# Autodesk Inventor assembly: ASSEMBLY_Main
(part 3 of 4)
- Równoległy:93 [Flush] (2 mm): COTS_GENERIC_20x40mm_alu_extrusion_560mm:1 ↔ LCBN_ALU_2mm_Y_Axis_Motor_Mount:1
- Zestawiający:100 [Mate]: COTS_GENERIC_Bearing_12x5x5:1 ↔ COTS_GENERIC_Y_Axis_Timing_Belt:1
- Zestawiający:101 [Mate]: COTS_GENERIC_NEMA23_Stepper_Motor:1 ↔ COTS_GENERIC_Y_Axis_Timing_Belt:1
- Zestawiający:102 [Mate] (0.5 mm): COTS_GENERIC_NEMA23_Stepper_Motor:1 ↔ COTS_GENERIC_Y_Axis_Timing_Belt:1
- Zestawiający:103 [Mate] (1 mm): COTS_GENERIC_Bearing_12x5x5:1 ↔ COTS_GENERIC_22x5_Washer:2
- Zestawiający:104 [Mate] (1 mm): COTS_GENERIC_Bearing_12x5x5:2 ↔ COTS_GENERIC_22x5_Washer:1
- Zestawiający:107 [Mate]: LCBN_ALU_3mm_Y_Axis_Idler_Stiffener_Top:1 ↔ COTS_GENERIC_22x5_Washer:2
- Zestawiający:108 [Mate]: LCBN_STEEL_3mm_Y_Axis_Heatbed_Baseplate:1 ↔ 3DP_ABS_Y_Axis_Linear_Bearing_Mount_Top:1
- Zestawiający:109 [Mate]: LCBN_STEEL_3mm_Y_Axis_Heatbed_Baseplate:1 ↔ 3DP_ABS_Y_Axis_Linear_Bearing_Mount_Top:4
- Zestawiający:110 [Mate]: LCBN_STEEL_3mm_Y_Axis_Heatbed_Baseplate:1 ↔ 3DP_ABS_Y_Axis_Linear_Bearing_Mount_Top:3
- Zestawiający:111 [Mate]: LCBN_STEEL_3mm_Y_Axis_Heatbed_Baseplate:1 ↔ 3DP_ABS_Y_Axis_Linear_Bearing_Mount_Top:2
- Zestawiający:112 [Mate]: LCBN_STEEL_3mm_Y_Axis_Heatbed_Baseplate:1 ↔ 3DP_ABS_Y_Axis_Linear_Bearing_Mount_Top:1
- Zestawiający:113 [Mate]: LCBN_STEEL_3mm_Y_Axis_Heatbed_Baseplate:1 ↔ 3DP_ABS_Y_Axis_Linear_Bearing_Mount_Top:1
- Zestawiający:114 [Mate]: LCBN_STEEL_3mm_Y_Axis_Heatbed_Baseplate:1 ↔ 3DP_ABS_Y_Axis_Linear_Bearing_Mount_Top:4
- Zestawiający:115 [Mate]: LCBN_STEEL_3mm_Y_Axis_Heatbed_Baseplate:1 ↔ 3DP_ABS_Y_Axis_Linear_Bearing_Mount_Top:4
- Zestawiający:116 [Mate]: LCBN_STEEL_3mm_Y_Axis_Heatbed_Baseplate:1 ↔ 3DP_ABS_Y_Axis_Linear_Bearing_Mount_Top:3
- Zestawiający:117 [Mate]: LCBN_STEEL_3mm_Y_Axis_Heatbed_Baseplate:1 ↔ 3DP_ABS_Y_Axis_Linear_Bearing_Mount_Top:3
- Zestawiający:118 [Mate]: LCBN_STEEL_3mm_Y_Axis_Heatbed_Baseplate:1 ↔ 3DP_ABS_Y_Axis_Linear_Bearing_Mount_Top:2
- Zestawiający:119 [Mate]: LCBN_STEEL_3mm_Y_Axis_Heatbed_Baseplate:1 ↔ 3DP_ABS_Y_Axis_Linear_Bearing_Mount_Top:2
- Zestawiający:120 [Mate] (1 mm): 3DP_ABS_Y_Axis_Linear_Bearing_Mount_Top:3 ↔ 3DP_ABS_Y_Axis_Linear_Bearing_Mount_Bottom:1
- Zestawiający:121 [Mate] (1 mm): 3DP_ABS_Y_Axis_Linear_Bearing_Mount_Top:2 ↔ 3DP_ABS_Y_Axis_Linear_Bearing_Mount_Bottom:3
- Zestawiający:122 [Mate] (1 mm): 3DP_ABS_Y_Axis_Linear_Bearing_Mount_Top:4 ↔ 3DP_ABS_Y_Axis_Linear_Bearing_Mount_Bottom:2
- Zestawiający:123 [Mate] (1 mm): 3DP_ABS_Y_Axis_Linear_Bearing_Mount_Top:1 ↔ 3DP_ABS_Y_Axis_Linear_Bearing_Mount_Bottom:4
- Równoległy:94 [Flush]: 3DP_ABS_Y_Axis_Linear_Bearing_Mount_Top:1 ↔ 3DP_ABS_Y_Axis_Linear_Bearing_Mount_Bottom:4
- Równoległy:95 [Flush] (3 mm): 3DP_ABS_Y_Axis_Linear_Bearing_Mount_Top:1 ↔ 3DP_ABS_Y_Axis_Linear_Bearing_Mount_Bottom:4
- Równoległy:96 [Flush]: 3DP_ABS_Y_Axis_Linear_Bearing_Mount_Top:4 ↔ 3DP_ABS_Y_Axis_Linear_Bearing_Mount_Bottom:2
- Równoległy:97 [Flush] (3 mm): 3DP_ABS_Y_Axis_Linear_Bearing_Mount_Top:4 ↔ 3DP_ABS_Y_Axis_Linear_Bearing_Mount_Bottom:2
- Równoległy:98 [Flush]: 3DP_ABS_Y_Axis_Linear_Bearing_Mount_Top:2 ↔ 3DP_ABS_Y_Axis_Linear_Bearing_Mount_Bottom:3
- Równoległy:99 [Flush] (3 mm): 3DP_ABS_Y_Axis_Linear_Bearing_Mount_Top:2 ↔ 3DP_ABS_Y_Axis_Linear_Bearing_Mount_Bottom:3
- Równoległy:100 [Flush]: 3DP_ABS_Y_Axis_Linear_Bearing_Mount_Top:3 ↔ 3DP_ABS_Y_Axis_Linear_Bearing_Mount_Bottom:1
- Równoległy:101 [Flush] (3 mm): 3DP_ABS_Y_Axis_Linear_Bearing_Mount_Top:3 ↔ 3DP_ABS_Y_Axis_Linear_Bearing_Mount_Bottom:1
- Zestawiający:124 [Mate]: COTS_GENERIC_LM10UU_10mm_Linear_Bearing:3 ↔ 3DP_ABS_Y_Axis_Linear_Bearing_Mount_Top:2
- Zestawiający:125 [Mate]: CUT_STEEL_10mmx457mm_Linear_Shaft:2 ↔ 3DP_ABS_Y_Axis_Linear_Bearing_Mount_Top:4
- Zestawiający:126 [Mate] (0.25 mm): COTS_GENERIC_LM10UU_10mm_Linear_Bearing:2 ↔ 3DP_ABS_Y_Axis_Linear_Bearing_Mount_Top:4
- Zestawiający:127 [Mate] (0.25 mm): COTS_GENERIC_LM10UU_10mm_Linear_Bearing:3 ↔ 3DP_ABS_Y_Axis_Linear_Bearing_Mount_Top:2
- Zestawiający:128 [Mate] (0.25 mm): COTS_GENERIC_LM10UU_10mm_Linear_Bearing:1 ↔ 3DP_ABS_Y_Axis_Linear_Bearing_Mount_Top:1
- Zestawiający:129 [Mate] (0.25 mm): COTS_GENERIC_LM10UU_10mm_Linear_Bearing:4 ↔ 3DP_ABS_Y_Axis_Linear_Bearing_Mount_Top:3
- Zestawiający:130 [Mate]: LCBN_STEEL_3mm_Y_Axis_Heatbed_Baseplate:1 ↔ 3DP_ABS_Y_Axis_Belt_Mount_Spacer:1
- Zestawiający:131 [Mate]: LCBN_STEEL_3mm_Y_Axis_Heatbed_Baseplate:1 ↔ 3DP_ABS_Y_Axis_Belt_Mount_Spacer:2
- Zestawiający:132 [Mate]: LCBN_STEEL_3mm_Y_Axis_Heatbed_Baseplate:1 ↔ 3DP_ABS_Y_Axis_Belt_Mount_Spacer:1
- Zestawiający:133 [Mate]: LCBN_STEEL_3mm_Y_Axis_Heatbed_Baseplate:1 ↔ 3DP_ABS_Y_Axis_Belt_Mount_Spacer:2
- Równoległy:102 [Flush] (2.5 mm): LCBN_STEEL_3mm_Y_Axis_Heatbed_Baseplate:1 ↔ 3DP_ABS_Y_Axis_Belt_Mount_Spacer:1
- Równoległy:103 [Flush] (2.5 mm): LCBN_STEEL_3mm_Y_Axis_Heatbed_Baseplate:1 ↔ 3DP_ABS_Y_Axis_Belt_Mount_Spacer:2
- Zestawiający:134 [Mate]: COTS_GENERIC_SMA12GUU_Linear_Bearing_Block:2 ↔ LC_ALU_4mm_X_End_Motor_Side:1
- Zestawiający:135 [Mate] (3 mm): COTS_GENERIC_NEMA17_25mm_shaft:1 ↔ LC_ALU_4mm_X_End_Motor_Side:1
- Równoległy:104 [Flush]: COTS_GENERIC_SMA12GUU_Linear_Bearing_Block:2 ↔ LC_ALU_4mm_X_End_Motor_Side:1
- Równoległy:105 [Flush]: COTS_GENERIC_SMA12GUU_Linear_Bearing_Block:4 ↔ LC_ALU_4mm_X_End_Motor_Side:1
- Równoległy:106 [Flush]: COTS_GENERIC_SMA12GUU_Linear_Bearing_Block:2 ↔ LC_ALU_4mm_X_End_Motor_Side:1
- Zestawiający:137 [Mate]: LC_ALU_4mm_X_End_Motor_Side:1 ↔ 3DP_ABS_X_Axis_Linear_Shaft_Clamp_Base:1
- Zestawiający:138 [Mate]: LC_ALU_4mm_X_End_Motor_Side:1 ↔ 3DP_ABS_X_Axis_Linear_Shaft_Clamp_Base:2
- Równoległy:107 [Flush]: LC_ALU_4mm_X_End_Motor_Side:1 ↔ 3DP_ABS_X_Axis_Linear_Shaft_Clamp_Base:1
- Równoległy:108 [Flush]: LC_ALU_4mm_X_End_Motor_Side:1 ↔ 3DP_ABS_X_Axis_Linear_Shaft_Clamp_Base:1
- Równoległy:109 [Flush]: LC_ALU_4mm_X_End_Motor_Side:1 ↔ 3DP_ABS_X_Axis_Linear_Shaft_Clamp_Base:2
- Równoległy:110 [Flush]: LC_ALU_4mm_X_End_Motor_Side:1 ↔ 3DP_ABS_X_Axis_Linear_Shaft_Clamp_Base:2
- Zestawiający:139 [Mate]: CUT_STEEL_10mmx516mm_Linear_Shaft:1 ↔ 3DP_ABS_X_Axis_Linear_Shaft_Clamp_Base:2
- Zestawiający:140 [Mate]: CUT_STEEL_10mmx516mm_Linear_Shaft:2 ↔ 3DP_ABS_X_Axis_Linear_Shaft_Clamp_Base:1
- Równoległy:111 [Flush]: CUT_STEEL_10mmx516mm_Linear_Shaft:1 ↔ 3DP_ABS_X_Axis_Linear_Shaft_Clamp_Base:2
- Równoległy:112 [Flush]: CUT_STEEL_10mmx516mm_Linear_Shaft:2 ↔ 3DP_ABS_X_Axis_Linear_Shaft_Clamp_Base:1
- Zestawiający:141 [Mate]: ASSEMBLY_X_Axis_Carriage_and_Extruder_Belt_Gearbox:1 ↔ CUT_STEEL_10mmx516mm_Linear_Shaft:2
- Zestawiający:142 [Mate] (-12 mm): ASSEMBLY_X_Axis_Carriage_and_Extruder_Belt_Gearbox:1 ↔ CUT_STEEL_10mmx516mm_Linear_Shaft:1
- Zestawiający:143 [Mate]: COTS_GENERIC_SMA12GUU_Linear_Bearing_Block:3 ↔ LC_ALU_4mm_X_End_Bearing_Side:1
- Równoległy:113 [Flush]: COTS_GENERIC_SMA12GUU_Linear_Bearing_Block:1 ↔ LC_ALU_4mm_X_End_Bearing_Side:1
- Równoległy:114 [Flush]: COTS_GENERIC_SMA12GUU_Linear_Bearing_Block:1 ↔ LC_ALU_4mm_X_End_Bearing_Side:1
- Zestawiający:144 [Mate]: LC_ALU_4mm_X_End_Bearing_Side:1 ↔ 3DP_ABS_X_Axis_Linear_Shaft_Clamp_Base:3
- Zestawiający:145 [Mate]: LC_ALU_4mm_X_End_Bearing_Side:1 ↔ 3DP_ABS_X_Axis_Linear_Shaft_Clamp_Base:4
- Równoległy:115 [Flush]: LC_ALU_4mm_X_End_Bearing_Side:1 ↔ 3DP_ABS_X_Axis_Linear_Shaft_Clamp_Base:4
- Równoległy:116 [Flush]: LC_ALU_4mm_X_End_Bearing_Side:1 ↔ 3DP_ABS_X_Axis_Linear_Shaft_Clamp_Base:3
- Równoległy:117 [Flush]: LC_ALU_4mm_X_End_Bearing_Side:1 ↔ 3DP_ABS_X_Axis_Linear_Shaft_Clamp_Base:4
- Równoległy:118 [Flush]: LC_ALU_4mm_X_End_Bearing_Side:1 ↔ 3DP_ABS_X_Axis_Linear_Shaft_Clamp_Base:3
- Zestawiający:146 [Mate] (1 mm): 3DP_ABS_X_Axis_Linear_Shaft_Clamp_Base:1 ↔ 3DP_ABS_X_Axis_Linear_Shaft_Clamp_Top:2
- Równoległy:119 [Flush]: 3DP_ABS_X_Axis_Linear_Shaft_Clamp_Base:1 ↔ 3DP_ABS_X_Axis_Linear_Shaft_Clamp_Top:2
- Równoległy:120 [Flush]: 3DP_ABS_X_Axis_Linear_Shaft_Clamp_Base:1 ↔ 3DP_ABS_X_Axis_Linear_Shaft_Clamp_Top:2
- Zestawiający:147 [Mate] (1 mm): 3DP_ABS_X_Axis_Linear_Shaft_Clamp_Base:3 ↔ 3DP_ABS_X_Axis_Linear_Shaft_Clamp_Top:1
- Równoległy:121 [Flush]: 3DP_ABS_X_Axis_Linear_Shaft_Clamp_Base:3 ↔ 3DP_ABS_X_Axis_Linear_Shaft_Clamp_Top:1
- Równoległy:122 [Flush]: 3DP_ABS_X_Axis_Linear_Shaft_Clamp_Base:3 ↔ 3DP_ABS_X_Axis_Linear_Shaft_Clamp_Top:1
- Zestawiający:149 [Mate]: 3DP_ABS_X_Axis_Linear_Shaft_Clamp_Base:4 ↔ 3DP_ABS_X_Axis_Linear_Shaft_Clamp_Bottom:2
- Równoległy:123 [Flush]: 3DP_ABS_X_Axis_Linear_Shaft_Clamp_Base:4 ↔ 3DP_ABS_X_Axis_Linear_Shaft_Clamp_Bottom:2
- Równoległy:124 [Flush]: 3DP_ABS_X_Axis_Linear_Shaft_Clamp_Base:4 ↔ 3DP_ABS_X_Axis_Linear_Shaft_Clamp_Bottom:2
- Zestawiający:152 [Mate]: COTS_GENERIC_20x40mm_alu_extrusion_460mm:1 ↔ 3DP_PLA_Controller_Case_Bottom:1
- Równoległy:128 [Flush]: COTS_GENERIC_20x40mm_alu_extrusion_560mm:1 ↔ 3DP_PLA_Controller_Case_Bottom:1
- Równoległy:129 [Flush]: COTS_GENERIC_20x40mm_alu_extrusion_460mm:1 ↔ 3DP_PLA_Controller_Case_Bottom:1
- Zestawiający:154 [Mate]: 3DP_PLA_Controller_Case_Bottom:1 ↔ 3DP_PLA_Controller_Case_Side_Wall_Longer:1
- Równoległy:130 [Flush]: 3DP_PLA_Controller_Case_Bottom:1 ↔ 3DP_PLA_Controller_Case_Side_Wall_Longer:1
- Równoległy:131 [Flush]: 3DP_PLA_Controller_Case_Bottom:1 ↔ 3DP_PLA_Controller_Case_Side_Wall_Longer:1
- Zestawiający:155 [Mate]: 3DP_PLA_Controller_Case_Bottom:1 ↔ 3DP_PLA_Controller_Case_Side_Wall_Shorter:1
- Równoległy:132 [Flush]: 3DP_PLA_Controller_Case_Bottom:1 ↔ 3DP_PLA_Controller_Case_Side_Wall_Shorter:1
- Równoległy:133 [Flush]: 3DP_PLA_Controller_Case_Bottom:1 ↔ 3DP_PLA_Controller_Case_Side_Wall_Shorter:1
- Zestawiający:156 [Mate]: COTS_GENERIC_RAMPS_14_Ardunio_Mega:1 ↔ 3DP_PLA_Controller_Case_Bottom:1
- Zestawiający:157 [Mate]: 3DP_PLA_Controller_Case_Side_Wall_Longer:1 ↔ 3DP_PLA_Controller_Case_Top:1
- Równoległy:134 [Flush]: COTS_GENERIC_20x40mm_alu_extrusion_460mm:1 ↔ 3DP_PLA_Controller_Case_Top:1
- Równoległy:135 [Flush]: COTS_GENERIC_20x40mm_alu_extrusion_560mm:1 ↔ 3DP_PLA_Controller_Case_Top:1
- Zestawiający:158 [Mate]: COTS_GENERIC_80mm_fan:1 ↔ 3DP_PLA_Controller_Case_Top:1
- Zestawiający:159 [Mate]: COTS_GENERIC_80mm_fan:1 ↔ 3DP_PLA_Controller_Case_Top:1
- Zestawiający:160 [Mate]: COTS_GENERIC_80mm_fan:1 ↔ 3DP_PLA_Controller_Case_Top:1
- Zestawiający:161 [Mate]: COTS_GENERIC_80mm_fan:1 ↔ 3DP_PLA_Controller_Case_Fan_Grill:1
- Zestawiający:162 [Mate]: COTS_GENERIC_80mm_fan:1 ↔ 3DP_PLA_Controller_Case_Fan_Grill:1
- Zestawiający:163 [Mate]: COTS_GENERIC_80mm_fan:1 ↔ 3DP_PLA_Controller_Case_Fan_Grill:1
- Zestawiający:164 [Mate]: COTS_GENERIC_20x40mm_alu_extrusion_560mm:2 ↔ 3DP_PLA_Filament_Spool_Rollers:2
- Zestawiający:165 [Mate]: COTS_GENERIC_20x40mm_alu_extrusion_560mm:2 ↔ 3DP_PLA_Filament_Spool_Rollers:1
- Równoległy:136 [Flush] (235 mm): COTS_GENERIC_20x40mm_alu_extrusion_460mm:3 ↔ 3DP_PLA_Filament_Spool_Rollers:1
- Zestawiający:166 [Mate] (1 mm): 3DP_PLA_Filament_Spool_Rollers:1 ↔ COTS_GENERIC_Bearing_19x5x6:1
- Zestawiający:167 [Mate] (1 mm): 3DP_PLA_Filament_Spool_Rollers:1 ↔ COTS_GENERIC_Bearing_19x5x6:2
- Zestawiający:168 [Mate] (1 mm): 3DP_PLA_Filament_Spool_Rollers:2 ↔ COTS_GENERIC_Bearing_19x5x6:4
- Zestawiający:169 [Mate] (1 mm): 3DP_PLA_Filament_Spool_Rollers:2 ↔ COTS_GENERIC_Bearing_19x5x6:3
- Zestawiający:170 [Mate]: 3DP_PLA_Filament_Spool_Rollers:1 ↔ COTS_GENERIC_Bearing_19x5x6:1
- Zestawiający:171 [Mate]: 3DP_PLA_Filament_Spool_Rollers:1 ↔ COTS_GENERIC_Bearing_19x5x6:2
- Zestawiający:172 [Mate]: 3DP_PLA_Filament_Spool_Rollers:2 ↔ COTS_GENERIC_Bearing_19x5x6:4
- Zestawiający:173 [Mate]: 3DP_PLA_Filament_Spool_Rollers:2 ↔ COTS_GENERIC_Bearing_19x5x6:3
- Zestawiający:174 [Mate] (-110.5 mm): COTS_GENERIC_Bearing_19x5x6:2 ↔ COTS_GENERIC_1_75mm_Filament_Spool:1
- Zestawiający:175 [Mate] (110.5 mm): COTS_GENERIC_Bearing_19x5x6:1 ↔ COTS_GENERIC_1_75mm_Filament_Spool:1
- Zestawiający:176 [Mate] (-10 mm): COTS_GENERIC_20x40mm_alu_extrusion_560mm:2 ↔ 3DP_PLA_Filament_Spool_Rollers:1
- Zestawiający:177 [Mate] (-10 mm): COTS_GENERIC_20x40mm_alu_extrusion_560mm:2 ↔ 3DP_PLA_Filament_Spool_Rollers:2
- Zestawiający:191 [Mate] (3.5 mm): COTS_GENERIC_RAMPS_14_Ardunio_Mega:1 ↔ 3DP_PLA_Controller_Case_Bottom:1
- Zestawiający:192 [Mate]: CUT_STEEL_10mmx516mm_Linear_Shaft:1 ↔ 3DP_ABS_X_Axis_Endstop_Mount:1
- Zestawiający:193 [Mate]: COTS_GENERIC_Endstop:2 ↔ 3DP_ABS_X_Axis_Endstop_Mount:1
- Równoległy:140 [Flush]: COTS_GENERIC_Endstop:2 ↔ 3DP_ABS_X_Axis_Endstop_Mount:1
- Równoległy:141 [Flush]: COTS_GENERIC_Endstop:2 ↔ 3DP_ABS_X_Axis_Endstop_Mount:1
- Równoległy:142 [Flush]: LC_ALU_4mm_X_End_Motor_Side:1 ↔ 3DP_ABS_X_Axis_Endstop_Mount:1
- Zestawiający:194 [Mate]: 3DP_ABS_X_Axis_Linear_Shaft_Clamp_Base:2 ↔ 3DP_ABS_X_Axis_Linear_Shaft_Clamp_Bottom_With_Endstop_Screw:1
- Równoległy:143 [Flush]: 3DP_ABS_X_Axis_Linear_Shaft_Clamp_Base:2 ↔ 3DP_ABS_X_Axis_Linear_Shaft_Clamp_Bottom_With_Endstop_Screw:1
- Równoległy:144 [Flush]: 3DP_ABS_X_Axis_Linear_Shaft_Clamp_Base:2 ↔ 3DP_ABS_X_Axis_Linear_Shaft_Clamp_Bottom_With_Endstop_Screw:1
- Zestawiający:197 [Mate]: 3DP_ABS_X_Axis_Linear_Shaft_Clamp_Bottom_With_Endstop_Screw:1 ↔ 3DP_ABS_Z_Axis_Screw_Nut_Mount:1
- Zestawiający:198 [Mate]: 3DP_ABS_X_Axis_Linear_Shaft_Clamp_Bottom:2 ↔ 3DP_ABS_Z_Axis_Screw_Nut_Mount:2
- Równoległy:145 [Flush]: 3DP_ABS_X_Axis_Linear_Shaft_Clamp_Bottom_With_Endstop_Screw:1 ↔ 3DP_ABS_Z_Axis_Screw_Nut_Mount:1
- Równoległy:146 [Flush]: 3DP_ABS_X_Axis_Linear_Shaft_Clamp_Bottom_With_Endstop_Screw:1 ↔ 3DP_ABS_Z_Axis_Screw_Nut_Mount:1
- Równoległy:147 [Flush]: 3DP_ABS_X_Axis_Linear_Shaft_Clamp_Bottom:2 ↔ 3DP_ABS_Z_Axis_Screw_Nut_Mount:2
- Równoległy:148 [Flush]: 3DP_ABS_X_Axis_Linear_Shaft_Clamp_Bottom:2 ↔ 3DP_ABS_Z_Axis_Screw_Nut_Mount:2
- Zestawiający:199 [Mate]: COTS_GENERIC_NEMA17_25mm_shaft:3 ↔ COTS_GENERIC_M6x350mm_Z_Axis_Screw:1
- Zestawiający:200 [Mate] (1 mm): COTS_GENERIC_NEMA17_25mm_shaft:3 ↔ COTS_GENERIC_M6x350mm_Z_Axis_Screw:1
- Zestawiający:201 [Mate]: COTS_GENERIC_NEMA17_25mm_shaft:2 ↔ COTS_GENERIC_M6x350mm_Z_Axis_Screw:2
- Zestawiający:202 [Mate] (1 mm): COTS_GENERIC_NEMA17_25mm_shaft:2 ↔ COTS_GENERIC_M6x350mm_Z_Axis_Screw:2
- Zestawiający:203 [Mate]: 3DP_ABS_Z_Axis_Screw_Nut_Mount:1 ↔ COTS_GENERIC_Z_Axis_M6_Screw_Nut:1
- Zestawiający:204 [Mate]: 3DP_ABS_Z_Axis_Screw_Nut_Mount:1 ↔ COTS_GENERIC_Z_Axis_M6_Screw_Nut:1
- Zestawiający:205 [Mate]: 3DP_ABS_Z_Axis_Screw_Nut_Mount:2 ↔ COTS_GENERIC_Z_Axis_M6_Screw_Nut:2
- Zestawiający:206 [Mate]: 3DP_ABS_Z_Axis_Screw_Nut_Mount:2 ↔ COTS_GENERIC_Z_Axis_M6_Screw_Nut:2
- Zestawiający:207 [Mate]: COTS_GENERIC_20x40mm_alu_extrusion_460mm:2 ↔ LC_ALU_4mm_Z_Axis_Motor_Mount:2
- Równoległy:149 [Flush]: COTS_GENERIC_20x40mm_alu_extrusion_460mm:2 ↔ LC_ALU_4mm_Z_Axis_Motor_Mount:2
- Zestawiający:208 [Mate]: COTS_GENERIC_NEMA17_25mm_shaft:2 ↔ LC_ALU_4mm_Z_Axis_Motor_Mount:2
- Zestawiający:211 [Mate]: COTS_GENERIC_20x40mm_alu_extrusion_460mm:1 ↔ LC_ALU_4mm_Z_Axis_Motor_Mount:1
- Równoległy:150 [Flush]: COTS_GENERIC_20x40mm_alu_extrusion_460mm:1 ↔ LC_ALU_4mm_Z_Axis_Motor_Mount:1
- Zestawiający:212 [Mate]: COTS_GENERIC_NEMA17_25mm_shaft:3 ↔ LC_ALU_4mm_Z_Axis_Motor_Mount:1
- Zestawiający:213 [Mate]: COTS_GENERIC_NEMA17_25mm_shaft:3 ↔ LC_ALU_4mm_Z_Axis_Motor_Mount:1
- Zestawiający:217 [Mate]: COTS_GENERIC_20x20mm_Angle_Bracket:5 ↔ LC_ALU_4mm_Z_Axis_Motor_Mount:2
- Zestawiający:218 [Mate]: COTS_GENERIC_20x20mm_Angle_Bracket:2 ↔ LC_ALU_4mm_Z_Axis_Motor_Mount:1
- Zestawiający:219 [Mate]: 3DP_ABS_Z_Axis_Screw_Nut_Mount:2 ↔ COTS_GENERIC_M6x350mm_Z_Axis_Screw:2
- Zestawiający:220 [Mate]: 3DP_ABS_Z_Axis_Screw_Nut_Mount:1 ↔ COTS_GENERIC_M6x350mm_Z_Axis_Screw:1
- Zestawiający:221 [Mate] (3 mm): 3DP_ABS_Z_Axis_Screw_Coupler:1 ↔ 3DP_ABS_Z_Axis_Screw_Coupler:4
- Zestawiający:222 [Mate] (3 mm): 3DP_ABS_Z_Axis_Screw_Coupler:2 ↔ 3DP_ABS_Z_Axis_Screw_Coupler:3
- Równoległy:151 [Flush]: 3DP_ABS_Z_Axis_Screw_Coupler:2 ↔ 3DP_ABS_Z_Axis_Screw_Coupler:3
- Równoległy:152 [Flush]: 3DP_ABS_Z_Axis_Screw_Coupler:2 ↔ 3DP_ABS_Z_Axis_Screw_Coupler:3
- Równoległy:153 [Flush]: 3DP_ABS_Z_Axis_Screw_Coupler:1 ↔ 3DP_ABS_Z_Axis_Screw_Coupler:4
- Równoległy:154 [Flush]: 3DP_ABS_Z_Axis_Screw_Coupler:1 ↔ 3DP_ABS_Z_Axis_Screw_Coupler:4
- Zestawiający:223 [Mate]: COTS_GENERIC_NEMA17_25mm_shaft:3 ↔ 3DP_ABS_Z_Axis_Screw_Coupler:3
- Zestawiający:224 [Mate]: COTS_GENERIC_NEMA17_25mm_shaft:2 ↔ 3DP_ABS_Z_Axis_Screw_Coupler:4
- Zestawiający:225 [Mate]: COTS_GENERIC_NEMA17_25mm_shaft:1 ↔ COTS_GENERIC_MXL_Pulley_X_Axis:1
- Zestawiający:226 [Mate] (2.5 mm): LC_ALU_4mm_X_End_Bearing_Side:1 ↔ COTS_GENERIC_Bearing_13x4x5:1
- Zestawiający:227 [Mate]: COTS_GENERIC_Bearing_13x4x5:1 ↔ COTS_GENERIC_Bearing_13x4x5:2
- Zestawiający:228 [Mate]: COTS_GENERIC_NEMA17_25mm_shaft:1 ↔ LC_ALU_4mm_X_End_Motor_Side:1
- Zestawiający:230 [Mate] (0.25 mm): COTS_GENERIC_20x40mm_alu_extrusion_460mm:3 ↔ 3DP_ABS_Cable_Pipe_Mount:2
- Zestawiający:231 [Mate] (0.25 mm): COTS_GENERIC_20x40mm_alu_extrusion_460mm:3 ↔ 3DP_ABS_Cable_Pipe_Mount:1
- Równoległy:155 [Flush] (100 mm): COTS_GENERIC_20x40mm_alu_extrusion_560mm:2 ↔ 3DP_ABS_Cable_Pipe_Mount:1
- Zestawiający:232 [Mate] (50 mm): COTS_GENERIC_20x40mm_alu_extrusion_460mm:1 ↔ 3DP_ABS_Cable_Pipe_Mount:2
- Zestawiający:233 [Mate]: COTS_GENERIC_20x40mm_alu_extrusion_460mm:3 ↔ 3DP_ABS_Cable_Pipe_Mount:2
- Zestawiający:234 [Mate]: COTS_GENERIC_20x40mm_alu_extrusion_460mm:3 ↔ 3DP_ABS_Cable_Pipe_Mount:1
- Zestawiający:236 [Mate]: COTS_GENERIC_Bearing_13x4x5:1 ↔ COTS_GENERIC_Bearing_13x4x5:2
- Zestawiający:237 [Mate]: LC_ALU_4mm_X_End_Bearing_Side:1 ↔ 3DP_ABS_X_End_Bearing_Mount:1
- Równoległy:156 [Flush] (1 mm): LC_ALU_4mm_X_End_Bearing_Side:1 ↔ 3DP_ABS_X_End_Bearing_Mount:1
- Równoległy:157 [Flush] (1 mm): LC_ALU_4mm_X_End_Bearing_Side:1 ↔ 3DP_ABS_X_End_Bearing_Mount:1
- Zestawiający:238 [Mate] (-10 mm): LC_ALU_4mm_X_End_Bearing_Side:1 ↔ COTS_GENERIC_Bearing_13x4x5:1
- Zestawiający:239 [Mate] (-10 mm): LC_ALU_4mm_X_End_Bearing_Side:1 ↔ COTS_GENERIC_Bearing_13x4x5:1
- Zestawiający:240 [Mate]: COTS_GENERIC_MXL_Pulley_X_Axis:1 ↔ COTS_GENERIC_X_Axis_Timing_Belt:1
- Zestawiający:241 [Mate] (0.5 mm): COTS_GENERIC_MXL_Pulley_X_Axis:1 ↔ COTS_GENERIC_X_Axis_Timing_Belt:1
- Równoległy:158 [Flush] (38.4 mm): COTS_GENERIC_SMA12GUU_Linear_Bearing_Block:2 ↔ COTS_GENERIC_X_Axis_Timing_Belt:1
- Zestawiający:242 [Mate] (0.5 mm): COTS_GENERIC_NEMA17_25mm_shaft:1 ↔ COTS_GENERIC_MXL_Pulley_X_Axis:1
- Zestawiający:243 [Mate]: COTS_GENERIC_NEMA17_25mm_shaft:1 ↔ 3DP_ABS_X_Axis_Motor_Spacer:1
- Równoległy:159 [Flush]: COTS_GENERIC_NEMA17_25mm_shaft:1 ↔ 3DP_ABS_X_Axis_Motor_Spacer:1
- Równoległy:160 [Flush]: COTS_GENERIC_NEMA17_25mm_shaft:1 ↔ 3DP_ABS_X_Axis_Motor_Spacer:1
- Mate:244: 3DP_ABS_X_Axis_Linear_Shaft_Clamp_Top:2 ↔ DIN 125-1 A A 5,3:1
- Mate:245: 3DP_ABS_X_Axis_Linear_Shaft_Clamp_Top:2 ↔ DIN 125-1 A A 5,3:1
- Mate:246: 3DP_ABS_X_Axis_Linear_Shaft_Clamp_Top:2 ↔ DIN 125-1 A A 5,3:2
- Mate:247: 3DP_ABS_X_Axis_Linear_Shaft_Clamp_Top:2 ↔ DIN 125-1 A A 5,3:2
- Mate:248: 3DP_ABS_X_Axis_Linear_Shaft_Clamp_Top:2 ↔ DIN 125-1 A A 5,3:3
- Mate:249: 3DP_ABS_X_Axis_Linear_Shaft_Clamp_Top:2 ↔ DIN 125-1 A A 5,3:3
- Mate:250: 3DP_ABS_X_Axis_Linear_Shaft_Clamp_Top:2 ↔ DIN 125-1 A A 5,3:4
- Mate:251: 3DP_ABS_X_Axis_Linear_Shaft_Clamp_Top:2 ↔ DIN 125-1 A A 5,3:4
- Mate:252: 3DP_ABS_X_Axis_Linear_Shaft_Clamp_Bottom_With_Endstop_Screw:1 ↔ DIN 125-1 A A 5,3:5
- Mate:253: 3DP_ABS_X_Axis_Linear_Shaft_Clamp_Top:2 ↔ DIN 125-1 A A 5,3:5
- Mate:254: 3DP_ABS_X_Axis_Linear_Shaft_Clamp_Bottom_With_Endstop_Screw:1 ↔ DIN 125-1 A A 5,3:6
- Mate:255: 3DP_ABS_X_Axis_Linear_Shaft_Clamp_Top:2 ↔ DIN 125-1 A A 5,3:6
- Mate:256: 3DP_ABS_X_Axis_Linear_Shaft_Clamp_Top:1 ↔ DIN 125-1 A A 5,3:7
- Mate:257: 3DP_ABS_X_Axis_Linear_Shaft_Clamp_Top:2 ↔ DIN 125-1 A A 5,3:7
- Mate:258: 3DP_ABS_X_Axis_Linear_Shaft_Clamp_Top:1 ↔ DIN 125-1 A A 5,3:8
- Mate:259: 3DP_ABS_X_Axis_Linear_Shaft_Clamp_Top:2 ↔ DIN 125-1 A A 5,3:8
- Mate:260: 3DP_ABS_X_Axis_Linear_Shaft_Clamp_Top:1 ↔ DIN 125-1 A A 5,3:9
- Mate:261: 3DP_ABS_X_Axis_Linear_Shaft_Clamp_Top:2 ↔ DIN 125-1 A A 5,3:9
- Mate:262: 3DP_ABS_X_Axis_Linear_Shaft_Clamp_Top:1 ↔ DIN 125-1 A A 5,3:10
- Mate:263: 3DP_ABS_X_Axis_Linear_Shaft_Clamp_Top:2 ↔ DIN 125-1 A A 5,3:10
- Mate:264: 3DP_ABS_X_Axis_Linear_Shaft_Clamp_Bottom:2 ↔ DIN 125-1 A A 5,3:11
- Mate:265: 3DP_ABS_X_Axis_Linear_Shaft_Clamp_Top:2 ↔ DIN 125-1 A A 5,3:11
- Mate:266: 3DP_ABS_X_Axis_Linear_Shaft_Clamp_Bottom:2 ↔ DIN 125-1 A A 5,3:12
- Mate:267: 3DP_ABS_X_Axis_Linear_Shaft_Clamp_Top:2 ↔ DIN 125-1 A A 5,3:12
- Insert:1: DIN 912 - replaced by DIN EN ISO 4762 M5 x 30:1 ↔ DIN 125-1 A A 5,3:1
- Insert:2: DIN 912 - replaced by DIN EN ISO 4762 M5 x 30:2 ↔ DIN 125-1 A A 5,3:2
- Insert:3: DIN 912 - replaced by DIN EN ISO 4762 M5 x 30:3 ↔ DIN 125-1 A A 5,3:3
- Insert:4: DIN 912 - replaced by DIN EN ISO 4762 M5 x 30:4 ↔ DIN 125-1 A A 5,3:4
- Insert:5: DIN 912 - replaced by DIN EN ISO 4762 M5 x 30:5 ↔ DIN 125-1 A A 5,3:5
- Insert:6: DIN 912 - replaced by DIN EN ISO 4762 M5 x 30:6 ↔ DIN 125-1 A A 5,3:6
- Insert:7: DIN 912 - replaced by DIN EN ISO 4762 M5 x 30:7 ↔ DIN 125-1 A A 5,3:7
- Insert:8: DIN 912 - replaced by DIN EN ISO 4762 M5 x 30:8 ↔ DIN 125-1 A A 5,3:8
- Insert:9: DIN 912 - replaced by DIN EN ISO 4762 M5 x 30:9 ↔ DIN 125-1 A A 5,3:9
- Insert:10: DIN 912 - replaced by DIN EN ISO 4762 M5 x 30:10 ↔ DIN 125-1 A A 5,3:10
- Insert:11: DIN 912 - replaced by DIN EN ISO 4762 M5 x 30:11 ↔ DIN 125-1 A A 5,3:11
- Insert:12: DIN 912 - replaced by DIN EN ISO 4762 M5 x 30:12 ↔ DIN 125-1 A A 5,3:12
- Mate:268: 3DP_ABS_Z_Axis_Screw_Nut_Mount:1 ↔ DIN 125-1 A A 5,3:13
- Mate:269: 3DP_ABS_Z_Axis_Screw_Nut_Mount:1 ↔ DIN 125-1 A A 5,3:13
- Mate:270: 3DP_ABS_Z_Axis_Screw_Nut_Mount:1 ↔ DIN 125-1 A A 5,3:14
- Mate:271: 3DP_ABS_Z_Axis_Screw_Nut_Mount:1 ↔ DIN 125-1 A A 5,3:14
- Mate:272: 3DP_ABS_Z_Axis_Screw_Nut_Mount:2 ↔ DIN 125-1 A A 5,3:15
- Mate:273: 3DP_ABS_Z_Axis_Screw_Nut_Mount:1 ↔ DIN 125-1 A A 5,3:15
- Mate:274: 3DP_ABS_Z_Axis_Screw_Nut_Mount:2 ↔ DIN 125-1 A A 5,3:16
- Mate:275: 3DP_ABS_Z_Axis_Screw_Nut_Mount:1 ↔ DIN 125-1 A A 5,3:16
- Insert:13: DIN 912 - replaced by DIN EN ISO 4762 M5 x 50:1 ↔ DIN 125-1 A A 5,3:13
- Insert:14: DIN 912 - replaced by DIN EN ISO 4762 M5 x 50:2 ↔ DIN 125-1 A A 5,3:14
- Insert:15: DIN 912 - replaced by DIN EN ISO 4762 M5 x 50:3 ↔ DIN 125-1 A A 5,3:15
- Insert:16: DIN 912 - replaced by DIN EN ISO 4762 M5 x 50:4 ↔ DIN 125-1 A A 5,3:16
- Mate:276: LC_ALU_4mm_X_End_Motor_Side:1 ↔ DIN 125-1 A A 3,2:1
- Mate:277: LC_ALU_4mm_X_End_Motor_Side:1 ↔ DIN 125-1 A A 3,2:1
- Mate:278: LC_ALU_4mm_X_End_Motor_Side:1 ↔ DIN 125-1 A A 3,2:2
- Mate:279: LC_ALU_4mm_X_End_Motor_Side:1 ↔ DIN 125-1 A A 3,2:2
- Mate:280: LC_ALU_4mm_X_End_Motor_Side:1 ↔ DIN 125-1 A A 3,2:3
- Mate:281: LC_ALU_4mm_X_End_Motor_Side:1 ↔ DIN 125-1 A A 3,2:3
- Mate:282: LC_ALU_4mm_X_End_Motor_Side:1 ↔ DIN 125-1 A A 3,2:4
- Mate:283: LC_ALU_4mm_X_End_Motor_Side:1 ↔ DIN 125-1 A A 3,2:4
- Mate:284: 3DP_ABS_X_Axis_Motor_Spacer:1 ↔ DIN 125-1 A A 3,2:5
- Mate:285: LC_ALU_4mm_X_End_Motor_Side:1 ↔ DIN 125-1 A A 3,2:5
- Insert:17: ISO 7380-1 M3 x 12:1 ↔ DIN 125-1 A A 3,2:1
- Insert:18: ISO 7380-1 M3 x 12:2 ↔ DIN 125-1 A A 3,2:2
- Insert:19: ISO 7380-1 M3 x 12:3 ↔ DIN 125-1 A A 3,2:3
- Insert:20: ISO 7380-1 M3 x 12:4 ↔ DIN 125-1 A A 3,2:4
- Insert:21: ISO 7380-1 M3 x 12:5 ↔ DIN 125-1 A A 3,2:5
- Mate:286: COTS_GENERIC_Endstop:2 ↔ DIN 125-1 A A 3,2:6
- Mate:287: COTS_GENERIC_Endstop:2 ↔ DIN 125-1 A A 3,2:6
- Insert:22: ISO 7380-1 M3 x 30:1 ↔ DIN 125-1 A A 3,2:6
- Mate:288: COTS_GENERIC_Endstop:2 ↔ DIN 125-1 A A 3,2:7
- Mate:289: 3DP_ABS_X_Axis_Endstop_Mount:1 ↔ DIN 125-1 A A 3,2:7
- Insert:23: DIN 934 - replaced by DIN EN 24032/28673/28674 M3:1 ↔ DIN 125-1 A A 3,2:7
- Mate:290: COTS_GENERIC_Endstop:2 ↔ DIN 125-1 A A 3,2:8
- Mate:291: COTS_GENERIC_Endstop:2 ↔ DIN 125-1 A A 3,2:8
- Insert:24: ISO 7380-1 M3 x 20:1 ↔ DIN 125-1 A A 3,2:8
- Mate:292: COTS_GENERIC_Endstop:2 ↔ DIN 125-1 A A 3,2:9
- Mate:293: 3DP_ABS_X_Axis_Endstop_Mount:1 ↔ DIN 125-1 A A 3,2:9
- Insert:25: DIN 934 - replaced by DIN EN 24032/28673/28674 M3:2 ↔ DIN 125-1 A A 3,2:9
- Mate:294: 3DP_ABS_X_Axis_Linear_Shaft_Clamp_Bottom_With_Endstop_Screw:1 ↔ DIN 125-1 A A 3,2:10
- Mate:295: 3DP_ABS_X_Axis_Linear_Shaft_Clamp_Bottom_With_Endstop_Screw:1 ↔ DIN 125-1 A A 3,2:10
- Insert:26: DIN 912 - replaced by DIN EN ISO 4762 M3 x 20:1 ↔ DIN 125-1 A A 3,2:10
- Mate:296: 3DP_ABS_X_Axis_Linear_Shaft_Clamp_Bottom_With_Endstop_Screw:1 ↔ DIN 125-1 A A 3,2:11
- Mate:297: 3DP_ABS_X_Axis_Linear_Shaft_Clamp_Bottom_With_Endstop_Screw:1 ↔ DIN 125-1 A A 3,2:11
- Insert:27: DIN 934 - replaced by DIN EN 24032/28673/28674 M3:3 ↔ DIN 125-1 A A 3,2:11
- Mate:298: 3DP_ABS_X_End_Bearing_Mount:1 ↔ DIN 125-1 A A 4,3:1
- Mate:299: 3DP_ABS_X_End_Bearing_Mount:1 ↔ DIN 125-1 A A 4,3:1
- Mate:300: COTS_GENERIC_Bearing_13x4x5:2 ↔ DIN 125-1 A A 4,3:3
- Mate:301: 3DP_ABS_X_End_Bearing_Mount:1 ↔ DIN 125-1 A A 4,3:3
- Insert:28: DIN 912 - replaced by DIN EN ISO 4762 M4 x 30:1 ↔ DIN 125-1 A A 4,3:1
- Insert:29: DIN 912 - replaced by DIN EN ISO 4762 M4 x 30:2 ↔ DIN 125-1 A A 4,3:3
- Mate:302: 3DP_ABS_X_End_Bearing_Mount:1 ↔ DIN 125-1 A A 4,3:2
- Mate:303: LC_ALU_4mm_X_End_Bearing_Side:1 ↔ DIN 125-1 A A 4,3:2
- Mate:304: COTS_GENERIC_Bearing_13x4x5:2 ↔ DIN 125-1 A A 4,3:4
- Mate:305: LC_ALU_4mm_X_End_Bearing_Side:1 ↔ DIN 125-1 A A 4,3:4
- Insert:30: DIN 934 - replaced by DIN EN 24032/28673/28674 M4:1 ↔ DIN 125-1 A A 4,3:2
- Insert:31: DIN 934 - replaced by DIN EN 24032/28673/28674 M4:2 ↔ DIN 125-1 A A 4,3:4
- Mate:306: COTS_GENERIC_20x40mm_alu_extrusion_560mm:2 ↔ COTS_GENERIC_20x20_M3_Nut:1
- Mate:307 (0.1 mm): COTS_GENERIC_20x40mm_alu_extrusion_560mm:2 ↔ COTS_GENERIC_20x20_M3_Nut:1
- Mate:308: 3DP_PLA_Filament_Spool_Rollers:2 ↔ DIN 125-1 A A 3,2:12
- Mate:309: 3DP_PLA_Filament_Spool_Rollers:2 ↔ DIN 125-1 A A 3,2:12
- Insert:32: DIN 912 - replaced by DIN EN ISO 4762 M3 x 16:1 ↔ DIN 125-1 A A 3,2:12
- Mate:310: DIN 912 - replaced by DIN EN ISO 4762 M3 x 16:1 ↔ COTS_GENERIC_20x20_M3_Nut:1
- Mate:311 (77 mm): 3DP_PLA_Filament_Spool_Rollers:1 ↔ 3DP_PLA_Filament_Spool_Rollers:2
- Mate:312: COTS_GENERIC_Bearing_19x5x6:4 ↔ DIN 125-1 A A 5,3:17
- Mate:313: COTS_GENERIC_Bearing_19x5x6:4 ↔ DIN 125-1 A A 5,3:17
- Mate:314: COTS_GENERIC_Bearing_19x5x6:3 ↔ DIN 125-1 A A 5,3:19
- Mate:315: COTS_GENERIC_Bearing_19x5x6:4 ↔ DIN 125-1 A A 5,3:19
- Insert:33: DIN 912 - replaced by DIN EN ISO 4762 M5 x 25:1 ↔ DIN 125-1 A A 5,3:17
- Insert:34: DIN 912 - replaced by DIN EN ISO 4762 M5 x 25:2 ↔ DIN 125-1 A A 5,3:19
- Mate:316: COTS_GENERIC_Bearing_19x5x6:4 ↔ DIN 125-1 A A 5,3:18
- Mate:317: 3DP_PLA_Filament_Spool_Rollers:2 ↔ DIN 125-1 A A 5,3:18
- Mate:318: COTS_GENERIC_Bearing_19x5x6:3 ↔ DIN 125-1 A A 5,3:20
- Mate:319: 3DP_PLA_Filament_Spool_Rollers:2 ↔ DIN 125-1 A A 5,3:20
- Insert:35: DIN 934 - replaced by DIN EN 24032/28673/28674 M5:1 ↔ DIN 125-1 A A 5,3:18
- Insert:36: DIN 934 - replaced by DIN EN 24032/28673/28674 M5:2 ↔ DIN 125-1 A A 5,3:20
- Mate:320: COTS_GENERIC_Bearing_19x5x6:1 ↔ DIN 125-1 A A 5,3:21
- Mate:321: COTS_GENERIC_Bearing_19x5x6:1 ↔ DIN 125-1 A A 5,3:21
- Mate:322: COTS_GENERIC_Bearing_19x5x6:2 ↔ DIN 125-1 A A 5,3:23
- Mate:323: COTS_GENERIC_Bearing_19x5x6:1 ↔ DIN 125-1 A A 5,3:23
- Insert:37: DIN 912 - replaced by DIN EN ISO 4762 M5 x 25:3 ↔ DIN 125-1 A A 5,3:21
- Insert:38: DIN 912 - replaced by DIN EN ISO 4762 M5 x 25:4 ↔ DIN 125-1 A A 5,3:23
- Mate:324: COTS_GENERIC_Bearing_19x5x6:1 ↔ DIN 125-1 A A 5,3:22
- Mate:325: 3DP_PLA_Filament_Spool_Rollers:1 ↔ DIN 125-1 A A 5,3:22
- Mate:326: COTS_GENERIC_Bearing_19x5x6:2 ↔ DIN 125-1 A A 5,3:24
- Mate:327: 3DP_PLA_Filament_Spool_Rollers:1 ↔ DIN 125-1 A A 5,3:24
- Insert:39: DIN 934 - replaced by DIN EN 24032/28673/28674 M5:3 ↔ DIN 125-1 A A 5,3:22
- Insert:40: DIN 934 - replaced by DIN EN 24032/28673/28674 M5:4 ↔ DIN 125-1 A A 5,3:24
- Mate:328: LC_ALU_3mm_Top_Beam_Mounting_Bracket:3 ↔ DIN 125-1 A A 5,3:25
- Mate:329: LC_ALU_3mm_Top_Beam_Mounting_Bracket:3 ↔ DIN 125-1 A A 5,3:25
- Mate:330: LC_ALU_3mm_Top_Beam_Mounting_Bracket:3 ↔ DIN 125-1 A A 5,3:26
- Mate:331: LC_ALU_3mm_Top_Beam_Mounting_Bracket:3 ↔ DIN 125-1 A A 5,3:26
- Mate:332: LC_ALU_3mm_Top_Beam_Mounting_Bracket:3 ↔ DIN 125-1 A A 5,3:27
- Mate:333: LC_ALU_3mm_Top_Beam_Mounting_Bracket:3 ↔ DIN 125-1 A A 5,3:27
- Mate:334: LC_ALU_3mm_Top_Beam_Mounting_Bracket:3 ↔ DIN 125-1 A A 5,3:28
- Mate:335: LC_ALU_3mm_Top_Beam_Mounting_Bracket:3 ↔ DIN 125-1 A A 5,3:28
- Mate:336: LC_ALU_3mm_Top_Beam_Mounting_Bracket:3 ↔ DIN 125-1 A A 5,3:29
- Mate:337: LC_ALU_3mm_Top_Beam_Mounting_Bracket:3 ↔ DIN 125-1 A A 5,3:29
- Insert:41: DIN 912 - replaced by DIN EN ISO 4762 M5 x 8:1 ↔ DIN 125-1 A A 5,3:25
- Insert:42: DIN 912 - replaced by DIN EN ISO 4762 M5 x 8:2 ↔ DIN 125-1 A A 5,3:26
- Insert:43: DIN 912 - replaced by DIN EN ISO 4762 M5 x 8:3 ↔ DIN 125-1 A A 5,3:27
- Insert:44: DIN 912 - replaced by DIN EN ISO 4762 M5 x 8:4 ↔ DIN 125-1 A A 5,3:28
- Insert:45: DIN 912 - replaced by DIN EN ISO 4762 M5 x 8:5 ↔ DIN 125-1 A A 5,3:29
- Flush:161 (-20 mm): COTS_GENERIC_20x40mm_alu_extrusion_560mm:2
- Insert:46: DIN 912 - replaced by DIN EN ISO 4762 M5 x 8:6 ↔ DIN 125-1 A A 5,3:30
- Insert:47: DIN 912 - replaced by DIN EN ISO 4762 M5 x 8:7 ↔ DIN 125-1 A A 5,3:31
- Insert:48: DIN 912 - replaced by DIN EN ISO 4762 M5 x 8:8 ↔ DIN 125-1 A A 5,3:32
- Insert:49: DIN 912 - replaced by DIN EN ISO 4762 M5 x 8:9 ↔ DIN 125-1 A A 5,3:33
- Insert:50: DIN 912 - replaced by DIN EN ISO 4762 M5 x 8:10 ↔ DIN 125-1 A A 5,3:34
- Flush:162 (-280 mm): COTS_GENERIC_20x40mm_alu_extrusion_560mm:2
- Insert:51: DIN 912 - replaced by DIN EN ISO 4762 M5 x 8:11 ↔ DIN 125-1 A A 5,3:35
- Insert:52: DIN 912 - replaced by DIN EN ISO 4762 M5 x 8:12 ↔ DIN 125-1 A A 5,3:36
- Insert:53: DIN 912 - replaced by DIN EN ISO 4762 M5 x 8:13 ↔ DIN 125-1 A A 5,3:37
- Insert:54: DIN 912 - replaced by DIN EN ISO 4762 M5 x 8:14 ↔ DIN 125-1 A A 5,3:38
- Insert:55: DIN 912 - replaced by DIN EN ISO 4762 M5 x 8:15 ↔ DIN 125-1 A A 5,3:39
- Insert:56: DIN 912 - replaced by DIN EN ISO 4762 M5 x 8:16 ↔ DIN 125-1 A A 5,3:40
- Insert:57: DIN 912 - replaced by DIN EN ISO 4762 M5 x 8:17 ↔ DIN 125-1 A A 5,3:41
- Insert:58: DIN 912 - replaced by DIN EN ISO 4762 M5 x 8:18 ↔ DIN 125-1 A A 5,3:42
- Insert:59: DIN 912 - replaced by DIN EN ISO 4762 M5 x 8:19 ↔ DIN 125-1 A A 5,3:43
- Insert:60: DIN 912 - replaced by DIN EN ISO 4762 M5 x 8:20 ↔ DIN 125-1 A A 5,3:44
- Mate:363 (3 mm): COTS_GENERIC_20x40mm_alu_extrusion_560mm:2 ↔ COTS_GENERIC_SHF12_Linear_Rail_Mount:1
- Mate:364 (2.5 mm): COTS_GENERIC_20x40mm_alu_extrusion_560mm:2 ↔ COTS_GENERIC_SHF12_Linear_Rail_Mount:2
- Mate:365: COTS_GENERIC_SHF12_Linear_Rail_Mount:2 ↔ DIN 125-1 A A 5,3:45
- Mate:366: COTS_GENERIC_SHF12_Linear_Rail_Mount:2 ↔ DIN 125-1 A A 5,3:45
- Mate:367: COTS_GENERIC_SHF12_Linear_Rail_Mount:2 ↔ DIN 125-1 A A 5,3:46
- Mate:368: COTS_GENERIC_SHF12_Linear_Rail_Mount:2 ↔ DIN 125-1 A A 5,3:46
- Mate:369: COTS_GENERIC_SHF12_Linear_Rail_Mount:1 ↔ DIN 125-1 A A 5,3:47
- Mate:370: COTS_GENERIC_SHF12_Linear_Rail_Mount:2 ↔ DIN 125-1 A A 5,3:47
- Mate:371: COTS_GENERIC_SHF12_Linear_Rail_Mount:1 ↔ DIN 125-1 A A 5,3:48
- Mate:372: COTS_GENERIC_SHF12_Linear_Rail_Mount:2 ↔ DIN 125-1 A A 5,3:48
- Insert:61: DIN 912 - replaced by DIN EN ISO 4762 M5 x 12:1 ↔ DIN 125-1 A A 5,3:45
- Insert:62: DIN 912 - replaced by DIN EN ISO 4762 M5 x 12:2 ↔ DIN 125-1 A A 5,3:46
- Insert:63: DIN 912 - replaced by DIN EN ISO 4762 M5 x 12:3 ↔ DIN 125-1 A A 5,3:47
- Insert:64: DIN 912 - replaced by DIN EN ISO 4762 M5 x 12:4 ↔ DIN 125-1 A A 5,3:48
- Angle:10 (0 deg): LC_ALU_4mm_Z_Axis_Motor_Mount:1 ↔ 3DP_ABS_Z_Axis_Screw_Coupler:2
- Angle:11 (0 deg): LC_ALU_4mm_Z_Axis_Motor_Mount:2 ↔ 3DP_ABS_Z_Axis_Screw_Coupler:1
- Mate:385: 3DP_ABS_Cable_Pipe_Mount:2 ↔ DIN 125-1 A A 3,2:16
- Mate:386: 3DP_ABS_Cable_Pipe_Mount:2 ↔ DIN 125-1 A A 3,2:16
- Mate:387: 3DP_ABS_Cable_Pipe_Mount:1 ↔ DIN 125-1 A A 3,2:17
- Mate:388: 3DP_ABS_Cable_Pipe_Mount:2 ↔ DIN 125-1 A A 3,2:17
- Insert:65: DIN 912 - replaced by DIN EN ISO 4762 M3 x 8:1 ↔ DIN 125-1 A A 3,2:16
- Insert:66: DIN 912 - replaced by DIN EN ISO 4762 M3 x 8:2 ↔ DIN 125-1 A A 3,2:17
- Mate:391: 3DP_ABS_Cable_Pipe_Mount:1 ↔ DIN 125-1 A A 3,2:18
- Mate:392: 3DP_ABS_Cable_Pipe_Mount:1 ↔ DIN 125-1 A A 3,2:18
- Mate:393: 3DP_ABS_Cable_Pipe_Mount:2 ↔ DIN 125-1 A A 3,2:19
- Mate:394: 3DP_ABS_Cable_Pipe_Mount:1 ↔ DIN 125-1 A A 3,2:19
- Insert:67: DIN 912 - replaced by DIN EN ISO 4762 M3 x 8:3 ↔ DIN 125-1 A A 3,2:18
- Insert:68: DIN 912 - replaced by DIN EN ISO 4762 M3 x 8:4 ↔ DIN 125-1 A A 3,2:19
- Mate:401: 3DP_ABS_Z_Axis_Endstop_Mount:1 ↔ DIN 7991 M3x8:1
- Mate:402: 3DP_ABS_Z_Axis_Endstop_Mount:1 ↔ DIN 7991 M3x8:2
- Mate:403: 3DP_ABS_Z_Axis_Screw_Coupler:2 ↔ DIN 125-1 A A 3,2:20
- Mate:404: 3DP_ABS_Z_Axis_Screw_Coupler:2 ↔ DIN 125-1 A A 3,2:20
- Mate:405: 3DP_ABS_Z_Axis_Screw_Coupler:2 ↔ DIN 125-1 A A 3,2:22
- Mate:406: 3DP_ABS_Z_Axis_Screw_Coupler:2 ↔ DIN 125-1 A A 3,2:22
- Mate:407: 3DP_ABS_Z_Axis_Screw_Coupler:2 ↔ DIN 125-1 A A 3,2:23
- Mate:408: 3DP_ABS_Z_Axis_Screw_Coupler:2 ↔ DIN 125-1 A A 3,2:23
- Mate:409: 3DP_ABS_Z_Axis_Screw_Coupler:2 ↔ DIN 125-1 A A 3,2:24
- Mate:410: 3DP_ABS_Z_Axis_Screw_Coupler:2 ↔ DIN 125-1 A A 3,2:24
- Mate:411: 3DP_ABS_Z_Axis_Screw_Coupler:1 ↔ DIN 125-1 A A 3,2:25
- Mate:412: 3DP_ABS_Z_Axis_Screw_Coupler:2 ↔ DIN 125-1 A A 3,2:25
- Mate:413: 3DP_ABS_Z_Axis_Screw_Coupler:1 ↔ DIN 125-1 A A 3,2:26
- Mate:414: 3DP_ABS_Z_Axis_Screw_Coupler:2 ↔ DIN 125-1 A A 3,2:26
- Mate:415: 3DP_ABS_Z_Axis_Screw_Coupler:1 ↔ DIN 125-1 A A 3,2:27
- Mate:416: 3DP_ABS_Z_Axis_Screw_Coupler:2 ↔ DIN 125-1 A A 3,2:27
- Mate:417: 3DP_ABS_Z_Axis_Screw_Coupler:1 ↔ DIN 125-1 A A 3,2:28
- Mate:418: 3DP_ABS_Z_Axis_Screw_Coupler:2 ↔ DIN 125-1 A A 3,2:28
- Insert:69: ISO 7380-1 M3 x 20:2 ↔ DIN 125-1 A A 3,2:20
- Insert:70: ISO 7380-1 M3 x 20:3 ↔ DIN 125-1 A A 3,2:22
- Insert:71: ISO 7380-1 M3 x 20:4 ↔ DIN 125-1 A A 3,2:23
- Insert:72: ISO 7380-1 M3 x 20:5 ↔ DIN 125-1 A A 3,2:24
- Insert:73: ISO 7380-1 M3 x 20:6 ↔ DIN 125-1 A A 3,2:25
- Insert:74: ISO 7380-1 M3 x 20:7 ↔ DIN 125-1 A A 3,2:26
- Insert:75: ISO 7380-1 M3 x 20:8 ↔ DIN 125-1 A A 3,2:27
- Insert:76: ISO 7380-1 M3 x 20:9 ↔ DIN 125-1 A A 3,2:28
- Mate:419: 3DP_ABS_Z_Axis_Screw_Coupler:2 ↔ DIN 125-1 A A 3,2:21
- Mate:420: 3DP_ABS_Z_Axis_Screw_Coupler:3 ↔ DIN 125-1 A A 3,2:21
- Mate:421: 3DP_ABS_Z_Axis_Screw_Coupler:2 ↔ DIN 125-1 A A 3,2:29
- Mate:422: 3DP_ABS_Z_Axis_Screw_Coupler:3 ↔ DIN 125-1 A A 3,2:29
- Mate:423: 3DP_ABS_Z_Axis_Screw_Coupler:2 ↔ DIN 125-1 A A 3,2:30
- Mate:424: 3DP_ABS_Z_Axis_Screw_Coupler:3 ↔ DIN 125-1 A A 3,2:30
- Mate:425: 3DP_ABS_Z_Axis_Screw_Coupler:2 ↔ DIN 125-1 A A 3,2:31
- Mate:426: 3DP_ABS_Z_Axis_Screw_Coupler:3 ↔ DIN 125-1 A A 3,2:31
- Mate:427: 3DP_ABS_Z_Axis_Screw_Coupler:1 ↔ DIN 125-1 A A 3,2:32
- Mate:428: 3DP_ABS_Z_Axis_Screw_Coupler:3 ↔ DIN 125-1 A A 3,2:32
- Mate:429: 3DP_ABS_Z_Axis_Screw_Coupler:1 ↔ DIN 125-1 A A 3,2:33
- Mate:430: 3DP_ABS_Z_Axis_Screw_Coupler:3 ↔ DIN 125-1 A A 3,2:33
- Mate:431: 3DP_ABS_Z_Axis_Screw_Coupler:1 ↔ DIN 125-1 A A 3,2:34
- Mate:432: 3DP_ABS_Z_Axis_Screw_Coupler:3 ↔ DIN 125-1 A A 3,2:34
- Mate:433: 3DP_ABS_Z_Axis_Screw_Coupler:1 ↔ DIN 125-1 A A 3,2:35
- Mate:434: 3DP_ABS_Z_Axis_Screw_Coupler:3 ↔ DIN 125-1 A A 3,2:35
- Insert:77: DIN 934 - replaced by DIN EN 24032/28673/28674 M3:4 ↔ DIN 125-1 A A 3,2:21
- Insert:78: DIN 125-1 A A 3,2:29 ↔ DIN 934 - replaced by DIN EN 24032/28673/28674 M3:5
- Insert:79: DIN 125-1 A A 3,2:30 ↔ DIN 934 - replaced by DIN EN 24032/28673/28674 M3:6
- Insert:80: DIN 934 - replaced by DIN EN 24032/28673/28674 M3:7 ↔ DIN 125-1 A A 3,2:31
- Insert:81: DIN 934 - replaced by DIN EN 24032/28673/28674 M3:8 ↔ DIN 125-1 A A 3,2:32
- Insert:82: DIN 934 - replaced by DIN EN 24032/28673/28674 M3:9 ↔ DIN 125-1 A A 3,2:33
- Insert:83: DIN 934 - replaced by DIN EN 24032/28673/28674 M3:10 ↔ DIN 125-1 A A 3,2:34
- Insert:84: DIN 934 - replaced by DIN EN 24032/28673/28674 M3:11 ↔ DIN 125-1 A A 3,2:35
- Mate:435 (-15 mm): COTS_GENERIC_NEMA17_25mm_shaft:3 ↔ 3DP_ABS_Z_Axis_Screw_Coupler:2
- Mate:436 (-15 mm): COTS_GENERIC_NEMA17_25mm_shaft:2 ↔ 3DP_ABS_Z_Axis_Screw_Coupler:1
- Mate:437: LC_ALU_4mm_Z_Axis_Motor_Mount:2 ↔ DIN 125-1 A A 3,2:36
- Mate:438: LC_ALU_4mm_Z_Axis_Motor_Mount:2 ↔ DIN 125-1 A A 3,2:36
- Mate:439: LC_ALU_4mm_Z_Axis_Motor_Mount:2 ↔ DIN 125-1 A A 3,2:37
- Mate:440: LC_ALU_4mm_Z_Axis_Motor_Mount:2 ↔ DIN 125-1 A A 3,2:37
- Mate:441: LC_ALU_4mm_Z_Axis_Motor_Mount:2 ↔ DIN 125-1 A A 3,2:38
- Mate:442: LC_ALU_4mm_Z_Axis_Motor_Mount:2 ↔ DIN 125-1 A A 3,2:38
- Mate:443: LC_ALU_4mm_Z_Axis_Motor_Mount:2 ↔ DIN 125-1 A A 3,2:39
- Mate:444: LC_ALU_4mm_Z_Axis_Motor_Mount:2 ↔ DIN 125-1 A A 3,2:39
- Mate:445: LC_ALU_4mm_Z_Axis_Motor_Mount:1 ↔ DIN 125-1 A A 3,2:40
- Mate:446: LC_ALU_4mm_Z_Axis_Motor_Mount:2 ↔ DIN 125-1 A A 3,2:40
- Mate:447: LC_ALU_4mm_Z_Axis_Motor_Mount:1 ↔ DIN 125-1 A A 3,2:41
- Mate:448: LC_ALU_4mm_Z_Axis_Motor_Mount:2 ↔ DIN 125-1 A A 3,2:41
- Mate:449: LC_ALU_4mm_Z_Axis_Motor_Mount:1 ↔ DIN 125-1 A A 3,2:42
- Mate:450: LC_ALU_4mm_Z_Axis_Motor_Mount:2 ↔ DIN 125-1 A A 3,2:42
- Mate:451: LC_ALU_4mm_Z_Axis_Motor_Mount:1 ↔ DIN 125-1 A A 3,2:43
- Mate:452: LC_ALU_4mm_Z_Axis_Motor_Mount:2 ↔ DIN 125-1 A A 3,2:43
- Insert:85: DIN 912 - replaced by DIN EN ISO 4762 M3 x 8:5 ↔ DIN 125-1 A A 3,2:36
- Insert:86: DIN 125-1 A A 3,2:37 ↔ DIN 912 - replaced by DIN EN ISO 4762 M3 x 8:6
- Insert:87: DIN 125-1 A A 3,2:38 ↔ DIN 912 - replaced by DIN EN ISO 4762 M3 x 8:7
- Insert:88: DIN 125-1 A A 3,2:39 ↔ DIN 912 - replaced by DIN EN ISO 4762 M3 x 8:8
- Insert:89: DIN 125-1 A A 3,2:40 ↔ DIN 912 - replaced by DIN EN ISO 4762 M3 x 8:9
- Insert:90: DIN 125-1 A A 3,2:41 ↔ DIN 912 - replaced by DIN EN ISO 4762 M3 x 8:10
- Insert:91: DIN 125-1 A A 3,2:42 ↔ DIN 912 - replaced by DIN EN ISO 4762 M3 x 8:11
- Insert:92: DIN 125-1 A A 3,2:43 ↔ DIN 912 - replaced by DIN EN ISO 4762 M3 x 8:12
- Mate:453: 3DP_PLA_Controller_Case_Fan_Grill:1 ↔ DIN 125-1 A A 4,3:5
- Mate:454: 3DP_PLA_Controller_Case_Fan_Grill:1 ↔ DIN 125-1 A A 4,3:5
- Mate:455: 3DP_PLA_Controller_Case_Fan_Grill:1 ↔ DIN 125-1 A A 4,3:7